# Autodesk Inventor assembly: Linear Slide
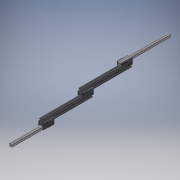
[picture p0: Inventor's stored thumbnail of the model, 180x180]
Saved by Autodesk Inventor 2017 (Build 210142000, 142)
## iProperties
Created: 2017-08-19
Part Number: Linear Slide
Document SubType Name: Assembly
Designer: slong
Author: slong
## Documents named in this file (5)
- C:\Users\slong\Desktop\ftc robot\linear slide\Linear Slide.iam
- C:\Users\slong\Desktop\ftc robot\linear slide\6760.iam
- C:\Users\slong\Desktop\ftc robot\linear slide\extruded aluminum linear slide.ipt
- C:\Users\slong\Desktop\ftc robot\extruded aluminum (vertical).ipt
- C:\Users\slong\Desktop\ftc robot\linear slide\1020-1-CL.ipt
## Components (16 placed, 4 different names)
1. 6760:1 [sub-assembly] — Mate:2, Flush:2, Flush:3, Flush:4, Flush:5, Mate:10
2. extruded aluminum (vertical):1 — Mate:2, Flush:2, Flush:3, Mate:3, Mate:5, Mate:7, Flush:7, Flush:27
3. 6760:2 [sub-assembly] — Mate:3, Flush:4, Flush:5, Mate:6
4. 6760:3 [sub-assembly] — Mate:5, Flush:6, Flush:7, Flush:8, Flush:9
5. extruded aluminum linear slide:2 — Mate:16, Flush:20, Mate:18, Flush:23, Flush:24, Mate:19, Flush:29
6. 1020-1-CL:1 — Flush:10, Mate:11, Mate:13, Flush:14, Flush:15, Mate:14, Mate:15, Flush:18, Flush:19, Mate:16, Flush:20, Mate:17, Flush:28, Flush:29
7. 1020-1-CL:2 — Mate:6, Mate:7, Flush:6, Mate:8, Flush:10, Mate:9, Flush:11, Mate:11, Mate:12, Flush:13, Flush:27, Flush:28
8. 6760:4 [sub-assembly] — Mate:8, Flush:8, Flush:9
9. 6760:5 [sub-assembly] — Mate:9, Mate:10, Flush:11, Flush:12
10. 6760:6 [sub-assembly] — Mate:12, Flush:12, Flush:13
11. 6760:7 [sub-assembly] — Mate:13, Flush:14, Flush:15, Flush:16, Flush:17
12. 6760:8 [sub-assembly] — Mate:14, Flush:16, Flush:17
13. 6760:9 [sub-assembly] — Mate:17, Flush:21, Flush:22
14. 6760:10 [sub-assembly] — Mate:15, Flush:18, Flush:19, Flush:21, Flush:22
15. 6760:11 [sub-assembly] — Mate:19, Flush:25, Flush:26
16. 6760:12 [sub-assembly] — Mate:18, Flush:23, Flush:24, Flush:25, Flush:26
## Relationships (45: Flush 28, Mate 17)
- Mate:2: 6760:1 ↔ extruded aluminum (vertical):1
- Flush:2: 6760:1 ↔ extruded aluminum (vertical):1
- Flush:3: 6760:1 ↔ extruded aluminum (vertical):1
- Mate:3: extruded aluminum (vertical):1 ↔ 6760:2
- Flush:4: 6760:1 ↔ 6760:2
- Mate:5 (0.1524 mm): extruded aluminum (vertical):1 ↔ 6760:3
- Flush:5: 6760:1 ↔ 6760:2
- Mate:6 (0.0127 mm): 6760:2 ↔ 1020-1-CL:2
- Mate:7 (4.2164 mm): extruded aluminum (vertical):1 ↔ 1020-1-CL:2
- Flush:6: 6760:3 ↔ 1020-1-CL:2
- Flush:7 (2.3876 mm): extruded aluminum (vertical):1 ↔ 6760:3
- Mate:8: 1020-1-CL:2 ↔ 6760:4
- Flush:8: 6760:3 ↔ 6760:4
- Flush:9: 6760:3 ↔ 6760:4
- Flush:10: 1020-1-CL:1 ↔ 1020-1-CL:2
- Mate:9: 1020-1-CL:2 ↔ 6760:5
- Mate:10 (2.413 mm): 6760:1 ↔ 6760:5
- Flush:11: 1020-1-CL:2 ↔ 6760:5
- Mate:11 (4.2164 mm): 1020-1-CL:1 ↔ 1020-1-CL:2
- Mate:12: 1020-1-CL:2 ↔ 6760:6
- Flush:12: 6760:5 ↔ 6760:6
- Flush:13: 1020-1-CL:2 ↔ 6760:6
- Mate:13: 1020-1-CL:1 ↔ 6760:7
- Flush:14 (25.4 mm): 1020-1-CL:1 ↔ 6760:7
- Flush:15: 1020-1-CL:1 ↔ 6760:7
- Mate:14: 1020-1-CL:1 ↔ 6760:8
- Flush:16: 6760:7 ↔ 6760:8
- Flush:17: 6760:7 ↔ 6760:8
- Mate:15: 1020-1-CL:1 ↔ 6760:10
- Flush:18 (25.4 mm): 1020-1-CL:1 ↔ 6760:10
- Flush:19: 1020-1-CL:1 ↔ 6760:10
- Mate:16 (4.2164 mm): extruded aluminum linear slide:2 ↔ 1020-1-CL:1
- Flush:20: extruded aluminum linear slide:2 ↔ 1020-1-CL:1
- Mate:17: 1020-1-CL:1 ↔ 6760:9
- Flush:21: 6760:9 ↔ 6760:10
- Flush:22: 6760:9 ↔ 6760:10
- Mate:18: extruded aluminum linear slide:2 ↔ 6760:12
- Flush:23: extruded aluminum linear slide:2 ↔ 6760:12
- Flush:24: extruded aluminum linear slide:2 ↔ 6760:12
- Mate:19: extruded aluminum linear slide:2 ↔ 6760:11
- Flush:25: 6760:11 ↔ 6760:12
- Flush:26: 6760:11 ↔ 6760:12
- Flush:27: extruded aluminum (vertical):1 ↔ 1020-1-CL:2
- Flush:28: 1020-1-CL:1 ↔ 1020-1-CL:2
- Flush:29: extruded aluminum linear slide:2 ↔ 1020-1-CL:1
